# Autodesk Inventor assembly: AssemblyRing7
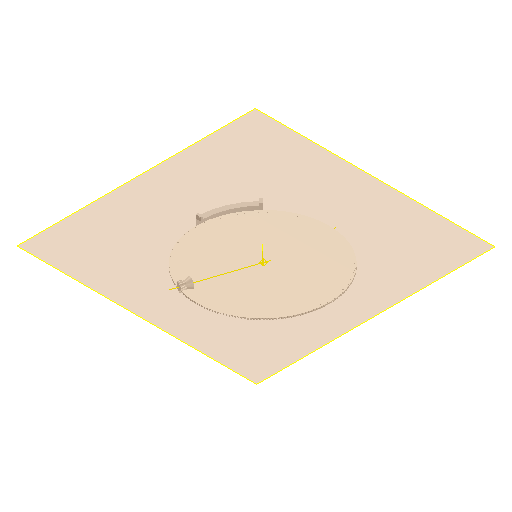
[picture p0: Inventor's stored thumbnail of the model, 512x512]
Saved by Autodesk Inventor 2022 (Build 260153000, 153)
## iProperties
Created: 2022-02-21
Part Number: AssemblyRing7
Document SubType Name: Assembly
Designer: lcroo
Author: lcroo
## Documents named in this file (4)
- C:\Users\32497\OneDrive - Vrije Universiteit Brussel\Documents\3BA\Bachelorproef\OneDrive_2022-04-19\Shared Folder\CAD\V7\Ring_Gear7.iam
- C:\Users\32497\OneDrive - Vrije Universiteit Brussel\Documents\3BA\Bachelorproef\OneDrive_2022-04-19\Shared Folder\CAD\V2\RingTanden.ipt
- C:\Users\32497\OneDrive - Vrije Universiteit Brussel\Documents\3BA\Bachelorproef\OneDrive_2022-04-19\Shared Folder\CAD\V2\AssemblyRing\Design Accelerator\Bevel Gears5.iam
- C:\Users\32497\OneDrive - Vrije Universiteit Brussel\Documents\3BA\Bachelorproef\OneDrive_2022-04-19\Shared Folder\CAD\V2\AssemblyRing\Design Accelerator\Bevel Gears8.iam
## Components (3 placed, 2 different names)
1. RingTanden:1 — Mate:1, Mate:2, Mate:3, Mate:4
2. Bevel Gears:2 [sub-assembly]
3. Bevel Gears:3 [sub-assembly] — Mate:3, Mate:4
## Relationships (5: Mate 4, Flush 1)
- Mate:1: RingTanden:1
- Mate:2: RingTanden:1
- Mate:3: RingTanden:1 ↔ Bevel Gears:3
- Mate:4: RingTanden:1 ↔ Bevel Gears:3
- Flush:1 (35 mm)
